# Autodesk Inventor assembly: MX-64T+idle.ipt_MIR
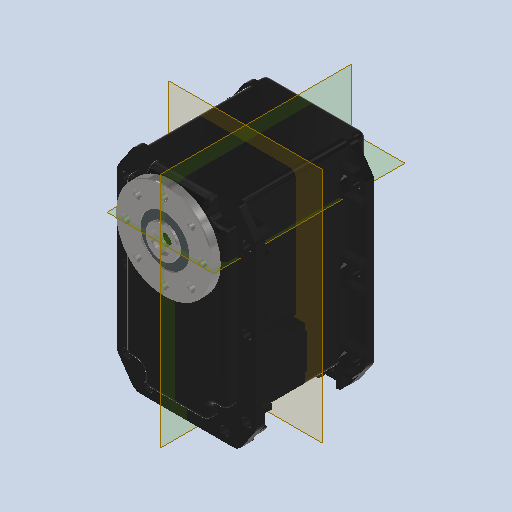
[picture p0: Inventor's stored thumbnail of the model, 512x512]
Saved by Autodesk Inventor 2024.3 (Build 283343000, 343)
## iProperties
Created: 2022-08-09
Part Number: MX-64T+idle.ipt_MIR
Document SubType Name: Assembly
Designer: gretc
Author: 박지훈
## Documents named in this file (3)
- C:\Users\gretc\Desktop\inventor_part\다이나믹셀\MX-64T+idle.ipt_MIR.iam
- C:\Users\gretc\Desktop\inventor_part\다이나믹셀\MX-64T_MIR.ipt
- C:\Users\gretc\Desktop\inventor_part\아이들러\64아이들러_MIR.iam
## Components (2 placed, 2 different names)
1. MX-64T_MIR:1 — 삽입:1
2. 64아이들러_MIR:1 [sub-assembly] — 삽입:1
## Relationships (1: Insert 1)
- 삽입:1 [Insert] (0.06 mm): MX-64T_MIR:1 ↔ 64아이들러_MIR:1
